# Autodesk Inventor assembly: Full Robot 1.1
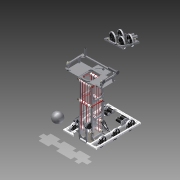
[picture p0: Inventor's stored thumbnail of the model, 180x180]
Saved by Autodesk Inventor 2011 SP1 (Build 150282100, 282)
## iProperties
Created: 2012-01-20
Part Number: Full Robot 1.1
Document SubType Name: Assembly
Designer: Christopher
Author: Christopher
## Documents named in this file (5)
- C:\Users\Christopher\Documents\Christopher\FIRST\Inventor files\2012\Full Robot 1.1.iam
- C:\Users\Christopher\Documents\Christopher\FIRST\Inventor files\2012\robot base.iam
- C:\Users\Christopher\Documents\Christopher\FIRST\Inventor files\2012\tower bottom second design\tower walls.ipt
- C:\Users\Christopher\Documents\Christopher\FIRST\Inventor files\2012\tower bottom second design\towerbottom2.5.iam
- C:\Users\Christopher\Documents\Christopher\FIRST\Inventor files\2012\4 wheel kicker version 1\game ball.ipt
## Components (4 placed, 4 different names)
1. robot base:1 [sub-assembly] — Mate:4, Mate:5, Mate:6, Mate:7
2. tower walls:1 — Mate:4
3. towerbottom2.5:1 [sub-assembly] — Mate:5, Mate:6, Mate:7
4. game ball:1
## Relationships (4: Mate 4)
- Mate:4 (88.9 mm): robot base:1 ↔ tower walls:1
- Mate:5: robot base:1 ↔ towerbottom2.5:1
- Mate:6: robot base:1 ↔ towerbottom2.5:1
- Mate:7 (101.6 mm): robot base:1 ↔ towerbottom2.5:1
